# Autodesk Inventor assembly: Ensamble de Prensa
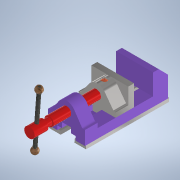
[picture p0: Inventor's stored thumbnail of the model, 180x180]
Saved by Autodesk Inventor 2021 (Build 250183000, 183)
## iProperties
Created: 2020-10-13
Part Number: Ensamble de Prensa
Document SubType Name: Assembly
Designer: IsaacFC
Author: IsaacFC
## Documents named in this file (17)
- E:\BILBAO\CADCAM\CADCAM 2021-1\PRENSA - copia\Ensamble de Prensa.iam
- E:\BILBAO\CADCAM\CADCAM 2021-1\PRENSA - copia\Pieza4_corredera_LAASR.ipt
- E:\BILBAO\CADCAM\CADCAM 2021-1\PRENSA - copia\09.TornilloSinFin.LPSM.ipt
- E:\BILBAO\CADCAM\CADCAM 2021-1\PRENSA - copia\1 Prisionero.ipt
- E:\BILBAO\CADCAM\CADCAM 2021-1\PRENSA - copia\Parte3_esfera.ipt
- E:\BILBAO\CADCAM\CADCAM 2021-1\PRENSA - copia\Parte5_BasePlaca_FMH.ipt
- E:\BILBAO\CADCAM\CADCAM 2021-1\PRENSA - copia\Pieza 10 RZ.ipt
- E:\BILBAO\CADCAM\CADCAM 2021-1\PRENSA - copia\Pieza7_tornillo.ipt
- E:\BILBAO\CADCAM\CADCAM 2021-1\PRENSA - copia\Eje.Proyecto 08.ipt
- E:\BILBAO\CADCAM\CADCAM 2021-1\PRENSA - copia\Parte2_Base.ipt
- E:\BILBAO\CADCAM\CADCAM 2021-1\PRENSA - copia\Parte 6_16ME.ipt
- E:\BILBAO\CADCAM\CADCAM 2021-1\PRENSA - copia\Ensamble de Prensa\AIP\FEA\de83b9icg.fins
- E:\BILBAO\CADCAM\CADCAM 2021-1\PRENSA - copia\Ensamble de Prensa\AIP\FEA\de83b9icg.fsat
- E:\BILBAO\CADCAM\CADCAM 2021-1\PRENSA - copia\Ensamble de Prensa\AIP\FEA\de83b9icg.ftes
- E:\BILBAO\CADCAM\CADCAM 2021-1\PRENSA - copia\Ensamble de Prensa\AIP\FEA\de83b9icg.fwiz
- E:\BILBAO\CADCAM\CADCAM 2021-1\PRENSA - copia\Ensamble de Prensa\AIP\FEA\de83b9ilc.fmsh
- E:\BILBAO\CADCAM\CADCAM 2021-1\PRENSA - copia\Ensamble de Prensa\AIP\FEA\de83b9ild.fres
## Components (16 placed, 10 different names)
1. Pieza4_corredera_LAASR:1 — Insert:1, Insert:2, Mate:1, Flush:1, Insert:15, Insert:16
2. 09.TornilloSinFin.LPSM:1 — Insert:1, Mate:2
3. 1 Prisionero:1 — Insert:2
4. Parte5_BasePlaca_FMH:1 — Insert:3, Insert:6, Insert:7, Insert:8
5. Parte5_BasePlaca_FMH:2 — Insert:4, Insert:5, Insert:9, Insert:10
6. Pieza 10 RZ:1 — Insert:9
7. Pieza 10 RZ:2 — Insert:10
8. Pieza 10 RZ:3 — Insert:7
9. Pieza 10 RZ:4 — Insert:8
10. Pieza7_tornillo:1 — Insert:18
11. Pieza7_tornillo:2 — Insert:17
12. Eje.Proyecto 08:1 — Mate:2, Insert:13, Insert:14
13. Parte2_Base:1 — Mate:1, Flush:1, Insert:3, Insert:4, Insert:5, Insert:6
14. Parte3_esfera:1 — Insert:14
15. Parte3_esfera:2 — Insert:13
16. Parte 6_16ME:1 — Insert:15, Insert:16, Insert:17, Insert:18
## Relationships (19: Insert 16, Mate 2, Flush 1)
- Insert:1 (1.5 mm): Pieza4_corredera_LAASR:1 ↔ 09.TornilloSinFin.LPSM:1
- Insert:2: Pieza4_corredera_LAASR:1 ↔ 1 Prisionero:1
- Mate:1: Pieza4_corredera_LAASR:1 ↔ Parte2_Base:1
- Flush:1: Pieza4_corredera_LAASR:1 ↔ Parte2_Base:1
- Mate:2: 09.TornilloSinFin.LPSM:1 ↔ Eje.Proyecto 08:1
- Insert:3: Parte5_BasePlaca_FMH:1 ↔ Parte2_Base:1
- Insert:4: Parte5_BasePlaca_FMH:2 ↔ Parte2_Base:1
- Insert:5: Parte5_BasePlaca_FMH:2 ↔ Parte2_Base:1
- Insert:6: Parte5_BasePlaca_FMH:1 ↔ Parte2_Base:1
- Insert:7: Parte5_BasePlaca_FMH:1 ↔ Pieza 10 RZ:3
- Insert:8: Parte5_BasePlaca_FMH:1 ↔ Pieza 10 RZ:4
- Insert:9: Parte5_BasePlaca_FMH:2 ↔ Pieza 10 RZ:1
- Insert:10: Parte5_BasePlaca_FMH:2 ↔ Pieza 10 RZ:2
- Insert:13: Eje.Proyecto 08:1 ↔ Parte3_esfera:2
- Insert:14: Eje.Proyecto 08:1 ↔ Parte3_esfera:1
- Insert:15: Pieza4_corredera_LAASR:1 ↔ Parte 6_16ME:1
- Insert:16: Pieza4_corredera_LAASR:1 ↔ Parte 6_16ME:1
- Insert:17: Pieza7_tornillo:2 ↔ Parte 6_16ME:1
- Insert:18: Pieza7_tornillo:1 ↔ Parte 6_16ME:1
## Named parameters: sa_0 = 0, sa_1 = 49050, sa_2 = 0
note: some values were not read from the file. Shown as the stored number, unit unknown: "sa_0", "sa_1", "sa_2".
